# Autodesk Inventor assembly: Full Assembly
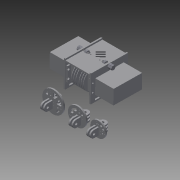
[picture p0: Inventor's stored thumbnail of the model, 180x180]
Saved by Autodesk Inventor 2014 SP1 (Build 180222100, 222)
## iProperties
Created: 2014-03-20
Part Number: Full Assembly
Document SubType Name: Assembly
Designer: ehagerup
Author: ehagerup
## Documents named in this file (5)
- C:\Users\ehagerup\SkyDrive\Documents\Mechanical Sketches\Animatronic Tail V4\Full Assembly.iam
- C:\Users\ehagerup\SkyDrive\Documents\Mechanical Sketches\Animatronic Tail V4\Assembly.iam
- C:\Users\ehagerup\SkyDrive\Documents\Mechanical Sketches\Animatronic Tail V4\Segment_Med_Ass.iam
- C:\Users\ehagerup\SkyDrive\Documents\Mechanical Sketches\Animatronic Tail V4\Segment_Small_Ass.iam
- C:\Users\ehagerup\SkyDrive\Documents\Mechanical Sketches\Animatronic Tail V4\Motor Assembly.iam
## Components (4 placed, 4 different names)
1. Assembly:1 [sub-assembly] — Flush:2, Flush:4
2. Segment_Med_Ass:1 [sub-assembly] — Flush:1, Flush:2, Flush:3, Flush:4
3. Segment_Small_Ass:1 [sub-assembly] — Flush:1, Flush:3
4. Motor Assembly:1 [sub-assembly]
## Relationships (4: Flush 4)
- Flush:1: Segment_Med_Ass:1 ↔ Segment_Small_Ass:1
- Flush:2: Assembly:1 ↔ Segment_Med_Ass:1
- Flush:3: Segment_Med_Ass:1 ↔ Segment_Small_Ass:1
- Flush:4: Assembly:1 ↔ Segment_Med_Ass:1
